# Autodesk Inventor assembly: Knee_LeftRear
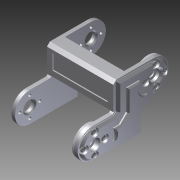
[picture p0: Inventor's stored thumbnail of the model, 180x180]
Saved by Autodesk Inventor 2015 (Build 190159000, 159)
## iProperties
Created: 2015-05-22
Part Number: Knee_LeftRear
Document SubType Name: Assembly
Designer: Quinn
Author: Quinn
## Documents named in this file (6)
- C:\Users\Quinn\Documents\GitHub\Project-Onyx-Quadruped\Local-Only\3DCNC Design\InventorModels\Assemblies\Knee_LeftRear.iam
- C:\Users\Quinn\Documents\GitHub\Project-Onyx-Quadruped\Local-Only\3DCNC Design\InventorModels\Electronics\Servo\ServoHornPlastic.ipt
- C:\Users\Quinn\Documents\GitHub\Project-Onyx-Quadruped\Local-Only\3DCNC Design\InventorModels\Assemblies\Knee_RightFront\Design Accelerator\Bolted Connection1.iam
- C:\Users\Quinn\Documents\GitHub\Project-Onyx-Quadruped\Local-Only\3DCNC Design\InventorModels\Assemblies\Knee_RightFront\Design Accelerator\Bolted Connection2.iam
- C:\Users\Quinn\Documents\GitHub\Project-Onyx-Quadruped\Local-Only\3DCNC Design\InventorModels\Assemblies\Knee_RightFront\Design Accelerator\Bolted Connection3.iam
- C:\Users\Quinn\Documents\GitHub\Project-Onyx-Quadruped\Local-Only\3DCNC Design\InventorModels\Plastics\KneeUpgradeMk3.1Blank.ipt
## Components (6 placed, 3 different names)
1. ServoHornPlastic:1 — Insert:1
2. ServoHornPlastic:2 — Insert:2, Mate:3, Mate:4
3. KneeUpgradeMk3.1Blank:1 — Insert:1, Insert:2, Mate:1, Mate:2, Mate:3, Mate:4, Mate:5, Mate:6, Mate:7, Mate:8
4. Bolted Connection:1 [sub-assembly] — Mate:1, Mate:2
5. Bolted Connection:2 [sub-assembly] — Mate:5, Mate:6
6. Bolted Connection:3 [sub-assembly] — Mate:7, Mate:8
## Relationships (10: Mate 8, Insert 2)
- Insert:1: ServoHornPlastic:1 ↔ KneeUpgradeMk3.1Blank:1
- Insert:2: ServoHornPlastic:2 ↔ KneeUpgradeMk3.1Blank:1
- Mate:1: KneeUpgradeMk3.1Blank:1 ↔ Bolted Connection:1
- Mate:2: KneeUpgradeMk3.1Blank:1 ↔ Bolted Connection:1
- Mate:3: ServoHornPlastic:2 ↔ KneeUpgradeMk3.1Blank:1
- Mate:4: ServoHornPlastic:2 ↔ KneeUpgradeMk3.1Blank:1
- Mate:5: KneeUpgradeMk3.1Blank:1 ↔ Bolted Connection:2
- Mate:6: KneeUpgradeMk3.1Blank:1 ↔ Bolted Connection:2
- Mate:7: KneeUpgradeMk3.1Blank:1 ↔ Bolted Connection:3
- Mate:8: KneeUpgradeMk3.1Blank:1 ↔ Bolted Connection:3
